# Autodesk Inventor assembly: assembly
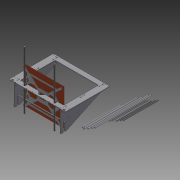
[picture p0: Inventor's stored thumbnail of the model, 180x180]
Saved by Autodesk Inventor 2013 (Build 170138000, 138)
## iProperties
Created: 2013-11-17
Part Number: assembly
Document SubType Name: Assembly
Designer: Masta
Author: Masta
## Documents named in this file (12)
- D:\prusa i3\frame\lasercut_aluminium\assembly.iam
- D:\prusa i3\frame\lasercut_aluminium\caddy.ipt
- D:\prusa i3\frame\lasercut_aluminium\main_frame.ipt
- D:\prusa i3\frame\lasercut_aluminium\side_frame.ipt
- D:\prusa i3\frame\lasercut_aluminium\fi8x320.ipt
- D:\prusa i3\frame\lasercut_aluminium\fi8x450.ipt
- D:\prusa i3\frame\lasercut_aluminium\fi8x470.ipt
- D:\prusa i3\frame\lasercut_aluminium\M5x300.ipt
- D:\prusa i3\frame\lasercut_aluminium\M8x290.ipt
- D:\prusa i3\frame\lasercut_aluminium\M8x410.ipt
- D:\prusa i3\frame\lasercut_aluminium\M10x480.ipt
- D:\prusa i3\frame\lasercut_aluminium\haetbed300.ipt
## Components (19 placed, 11 different names)
1. main_frame:1 — Mate:1, Flush:3, Mate:2, Mate:3, Mate:4, Flush:4, Insert:1, Insert:2
2. caddy:1 — Mate:4, Flush:4, Insert:4, Insert:5
3. side_frame:1 — Flush:1, Flush:2, Flush:3, Mate:3, Insert:3
4. side_frame:2 — Flush:1, Mate:1, Flush:2, Mate:2
5. fi8x320:1
6. fi8x320:2
7. fi8x450:1
8. fi8x450:2
9. fi8x470:1
10. fi8x470:2
11. M5x300:1
12. M5x300:2
13. M8x290:1
14. M8x290:2
15. M8x290:3
16. M8x410:1 — Insert:3
17. M10x480:1 — Insert:1
18. M10x480:2 — Insert:2
19. haetbed300:1 — Insert:4, Insert:5
## Relationships (13: Insert 5, Flush 4, Mate 4)
- Flush:1: side_frame:1 ↔ side_frame:2
- Mate:1: main_frame:1 ↔ side_frame:2
- Flush:2: side_frame:1 ↔ side_frame:2
- Flush:3: main_frame:1 ↔ side_frame:1
- Mate:2 (0.25 mm): main_frame:1 ↔ side_frame:2
- Mate:3 (0.25 mm): main_frame:1 ↔ side_frame:1
- Mate:4 (5 mm): main_frame:1 ↔ caddy:1
- Flush:4: main_frame:1 ↔ caddy:1
- Insert:1 (-200 mm): main_frame:1 ↔ M10x480:1
- Insert:2 (-200 mm): main_frame:1 ↔ M10x480:2
- Insert:3 (-11 mm): side_frame:1 ↔ M8x410:1
- Insert:4 (10 mm): caddy:1 ↔ haetbed300:1
- Insert:5 (10 mm): caddy:1 ↔ haetbed300:1
